# Autodesk Inventor assembly: HyperCube Evolution frame
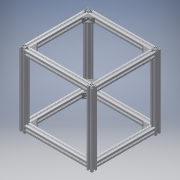
[picture p0: Inventor's stored thumbnail of the model, 180x180]
Saved by Autodesk Inventor 2016 (Build 200138000, 138)
## iProperties
Created: 2017-04-09
Part Number: HyperCube Evolution frame
Document SubType Name: Assembly
Designer: Scott
Author: Scott
## Documents named in this file (7)
- E:\Scott Projects\3D Printing\CoreXY\HyperCube Evolution frame.iam
- E:\Scott Projects\3D Printing\CoreXY\3030 Extrusion - X.ipt
- E:\Scott Projects\3D Printing\CoreXY\3030 Extrusion - Z.ipt
- E:\Scott Projects\3D Printing\CoreXY\3030 Extrusion - Y.ipt
- E:\Scott Projects\3D Printing\CoreXY\3030 Corner Bracket External.ipt
- C:\Users\Scott\Documents\Inventor\Content Center Files\R2016\en-US\ANSI B18.3.4M(1)\ANSI B18.3.4M - M5 x 0.8 x 10(2).ipt
- E:\Scott Projects\3D Printing\CoreXY\HyperCube parameters.xlsx
## Components (36 placed, 5 different names)
1. 3030 Extrusion - X:1 — Mate:1, Mate:2, Flush:1, Mate:4, Flush:2, Mate:5, Flush:7, Flush:13
2. 3030 Extrusion - Z:1 — Mate:3, Flush:1, Mate:4, Flush:3, Flush:5, Mate:9, Flush:10, Flush:11, Mate:10, Flush:12
3. 3030 Extrusion - Z:2 — Flush:2, Flush:3, Mate:5, Flush:4, Mate:6, Mate:7, Flush:6, Mate:8, Flush:8, Flush:9
4. 3030 Extrusion - X:2 — Flush:4, Mate:6, Flush:5, Mate:15, Flush:23, Mate:17
5. 3030 Extrusion - Y:1 — Mate:7, Flush:6, Flush:7, Flush:18, Flush:22
6. 3030 Extrusion - Y:2 — Mate:8, Flush:8, Flush:9, Mate:11, Flush:14, Flush:15, Flush:19, Mate:16, Mate:19
7. 3030 Extrusion - Y:3 — Mate:9, Flush:10, Flush:11, Mate:12, Flush:16, Flush:17, Mate:18, Mate:21
8. 3030 Extrusion - Y:4 — Mate:10, Flush:12, Flush:13
9. 3030 Extrusion - Z:3 — Mate:11, Flush:14, Flush:15, Mate:13, Flush:20, Mate:14, Flush:21
10. 3030 Extrusion - Z:4 — Mate:12, Flush:16, Flush:17
11. 3030 Extrusion - X:3 — Mate:13, Flush:19, Flush:20, Mate:20, Mate:22
12. 3030 Extrusion - X:4 — Mate:14, Flush:21, Flush:22
13. Broached Hexagon Socket Button Head Cap Screw - Metric M5 x 0.8 x 10:1 — Insert:2
14. Broached Hexagon Socket Button Head Cap Screw - Metric M5 x 0.8 x 10:2 — Insert:1
15. Broached Hexagon Socket Button Head Cap Screw - Metric M5 x 0.8 x 10:3 — Insert:4
16. Broached Hexagon Socket Button Head Cap Screw - Metric M5 x 0.8 x 10:4 — Insert:3
17. Broached Hexagon Socket Button Head Cap Screw - Metric M5 x 0.8 x 10:5 — Insert:5
18. Broached Hexagon Socket Button Head Cap Screw - Metric M5 x 0.8 x 10:6 — Insert:6
19. Broached Hexagon Socket Button Head Cap Screw - Metric M5 x 0.8 x 10:7 — Insert:8
20. Broached Hexagon Socket Button Head Cap Screw - Metric M5 x 0.8 x 10:8 — Insert:7
21. Broached Hexagon Socket Button Head Cap Screw - Metric M5 x 0.8 x 10:9 — Insert:10
22. Broached Hexagon Socket Button Head Cap Screw - Metric M5 x 0.8 x 10:10 — Insert:9
23. Broached Hexagon Socket Button Head Cap Screw - Metric M5 x 0.8 x 10:11 — Insert:12
24. Broached Hexagon Socket Button Head Cap Screw - Metric M5 x 0.8 x 10:12 — Insert:11
25. Broached Hexagon Socket Button Head Cap Screw - Metric M5 x 0.8 x 10:13 — Insert:13
26. Broached Hexagon Socket Button Head Cap Screw - Metric M5 x 0.8 x 10:14 — Insert:14
27. Broached Hexagon Socket Button Head Cap Screw - Metric M5 x 0.8 x 10:15 — Insert:16
28. Broached Hexagon Socket Button Head Cap Screw - Metric M5 x 0.8 x 10:16 — Insert:15
29. 3030 Corner Bracket External:2 — Mate:19, Mate:20, Flush:25, Insert:7, Insert:8
30. 3030 Corner Bracket External:1 — Mate:15, Mate:16, Flush:23, Flush:24, Flush:25, Insert:1, Insert:2
31. 3030 Corner Bracket External:4 — Mate:21, Mate:22, Flush:26, Insert:5, Insert:6
32. 3030 Corner Bracket External:3 — Mate:17, Mate:18, Flush:24, Flush:26, Insert:3, Insert:4
33. 3030 Corner Bracket External:5 — Insert:9, Insert:10
34. 3030 Corner Bracket External:6 — Insert:15, Insert:16
35. 3030 Corner Bracket External:7 — Insert:11, Insert:12
36. 3030 Corner Bracket External:8 — Insert:13, Insert:14
## Component patterns: (2 elements, first: 3030 Corner Bracket External:2 + 3030 Corner Bracket External:1 + 3030 Corner Bracket External:4 + 3030 Corner Bracket External:3)
## Relationships (64: Flush 26, Mate 22, Insert 16)
- Mate:1: 3030 Extrusion - X:1
- Mate:2 (10 mm): 3030 Extrusion - X:1
- Mate:3: 3030 Extrusion - Z:1
- Flush:1: 3030 Extrusion - X:1 ↔ 3030 Extrusion - Z:1
- Mate:4: 3030 Extrusion - X:1 ↔ 3030 Extrusion - Z:1
- Flush:2: 3030 Extrusion - X:1 ↔ 3030 Extrusion - Z:2
- Flush:3: 3030 Extrusion - Z:1 ↔ 3030 Extrusion - Z:2
- Mate:5: 3030 Extrusion - X:1 ↔ 3030 Extrusion - Z:2
- Flush:4: 3030 Extrusion - Z:2 ↔ 3030 Extrusion - X:2
- Mate:6: 3030 Extrusion - Z:2 ↔ 3030 Extrusion - X:2
- Flush:5: 3030 Extrusion - Z:1 ↔ 3030 Extrusion - X:2
- Mate:7: 3030 Extrusion - Z:2 ↔ 3030 Extrusion - Y:1
- Flush:6: 3030 Extrusion - Z:2 ↔ 3030 Extrusion - Y:1
- Flush:7: 3030 Extrusion - X:1 ↔ 3030 Extrusion - Y:1
- Mate:8: 3030 Extrusion - Z:2 ↔ 3030 Extrusion - Y:2
- Flush:8: 3030 Extrusion - Z:2 ↔ 3030 Extrusion - Y:2
- Flush:9: 3030 Extrusion - Z:2 ↔ 3030 Extrusion - Y:2
- Mate:9: 3030 Extrusion - Z:1 ↔ 3030 Extrusion - Y:3
- Flush:10: 3030 Extrusion - Z:1 ↔ 3030 Extrusion - Y:3
- Flush:11: 3030 Extrusion - Z:1 ↔ 3030 Extrusion - Y:3
- Mate:10: 3030 Extrusion - Z:1 ↔ 3030 Extrusion - Y:4
- Flush:12: 3030 Extrusion - Z:1 ↔ 3030 Extrusion - Y:4
- Flush:13: 3030 Extrusion - X:1 ↔ 3030 Extrusion - Y:4
- Mate:11: 3030 Extrusion - Y:2 ↔ 3030 Extrusion - Z:3
- Flush:14: 3030 Extrusion - Y:2 ↔ 3030 Extrusion - Z:3
- Flush:15: 3030 Extrusion - Y:2 ↔ 3030 Extrusion - Z:3
- Mate:12: 3030 Extrusion - Y:3 ↔ 3030 Extrusion - Z:4
- Flush:16: 3030 Extrusion - Y:3 ↔ 3030 Extrusion - Z:4
- Flush:17: 3030 Extrusion - Y:3 ↔ 3030 Extrusion - Z:4
- Flush:18: 3030 Extrusion - Y:1
- Mate:13: 3030 Extrusion - Z:3 ↔ 3030 Extrusion - X:3
- Flush:19: 3030 Extrusion - Y:2 ↔ 3030 Extrusion - X:3
- Flush:20: 3030 Extrusion - Z:3 ↔ 3030 Extrusion - X:3
- Mate:14: 3030 Extrusion - Z:3 ↔ 3030 Extrusion - X:4
- Flush:21: 3030 Extrusion - Z:3 ↔ 3030 Extrusion - X:4
- Flush:22: 3030 Extrusion - Y:1 ↔ 3030 Extrusion - X:4
- Mate:15: 3030 Extrusion - X:2 ↔ 3030 Corner Bracket External:1
- Mate:16: 3030 Extrusion - Y:2 ↔ 3030 Corner Bracket External:1
- Flush:23 (1 mm): 3030 Extrusion - X:2 ↔ 3030 Corner Bracket External:1
- Mate:17: 3030 Extrusion - X:2 ↔ 3030 Corner Bracket External:3
- Mate:18: 3030 Extrusion - Y:3 ↔ 3030 Corner Bracket External:3
- Flush:24: 3030 Corner Bracket External:1 ↔ 3030 Corner Bracket External:3
- Mate:19: 3030 Extrusion - Y:2 ↔ 3030 Corner Bracket External:2
- Mate:20: 3030 Extrusion - X:3 ↔ 3030 Corner Bracket External:2
- Flush:25: 3030 Corner Bracket External:2 ↔ 3030 Corner Bracket External:1
- Mate:21: 3030 Extrusion - Y:3 ↔ 3030 Corner Bracket External:4
- Mate:22: 3030 Extrusion - X:3 ↔ 3030 Corner Bracket External:4
- Flush:26: 3030 Corner Bracket External:4 ↔ 3030 Corner Bracket External:3
- Insert:1: Broached Hexagon Socket Button Head Cap Screw - Metric M5 x 0.8 x 10:2 ↔ 3030 Corner Bracket External:1
- Insert:2: Broached Hexagon Socket Button Head Cap Screw - Metric M5 x 0.8 x 10:1 ↔ 3030 Corner Bracket External:1
- Insert:3: Broached Hexagon Socket Button Head Cap Screw - Metric M5 x 0.8 x 10:4 ↔ 3030 Corner Bracket External:3
- Insert:4: Broached Hexagon Socket Button Head Cap Screw - Metric M5 x 0.8 x 10:3 ↔ 3030 Corner Bracket External:3
- Insert:5: Broached Hexagon Socket Button Head Cap Screw - Metric M5 x 0.8 x 10:5 ↔ 3030 Corner Bracket External:4
- Insert:6: Broached Hexagon Socket Button Head Cap Screw - Metric M5 x 0.8 x 10:6 ↔ 3030 Corner Bracket External:4
- Insert:7: Broached Hexagon Socket Button Head Cap Screw - Metric M5 x 0.8 x 10:8 ↔ 3030 Corner Bracket External:2
- Insert:8: Broached Hexagon Socket Button Head Cap Screw - Metric M5 x 0.8 x 10:7 ↔ 3030 Corner Bracket External:2
- Insert:9: Broached Hexagon Socket Button Head Cap Screw - Metric M5 x 0.8 x 10:10 ↔ 3030 Corner Bracket External:5
- Insert:10: Broached Hexagon Socket Button Head Cap Screw - Metric M5 x 0.8 x 10:9 ↔ 3030 Corner Bracket External:5
- Insert:11: Broached Hexagon Socket Button Head Cap Screw - Metric M5 x 0.8 x 10:12 ↔ 3030 Corner Bracket External:7
- Insert:12: Broached Hexagon Socket Button Head Cap Screw - Metric M5 x 0.8 x 10:11 ↔ 3030 Corner Bracket External:7
- Insert:13: Broached Hexagon Socket Button Head Cap Screw - Metric M5 x 0.8 x 10:13 ↔ 3030 Corner Bracket External:8
- Insert:14: Broached Hexagon Socket Button Head Cap Screw - Metric M5 x 0.8 x 10:14 ↔ 3030 Corner Bracket External:8
- Insert:15: Broached Hexagon Socket Button Head Cap Screw - Metric M5 x 0.8 x 10:16 ↔ 3030 Corner Bracket External:6
- Insert:16: Broached Hexagon Socket Button Head Cap Screw - Metric M5 x 0.8 x 10:15 ↔ 3030 Corner Bracket External:6
## Named parameters: frame_height = 400 mm, frame_depth = 380 mm, extrusion_size = 30 mm, frame_width = 400 mm, hole_spacing_depth = 210 mm, hole_spacing_width = 210 mm, platform_width = 214 mm, platform_depth = 214 mm, bed_frame_depth = 310 mm, bed_frame_width = 180 mm, bed_extrusion_size = 20 mm, bed_cl_y_offset = 173.25 mm, T8_screw_length = 250 mm
